# Autodesk Inventor assembly: gearLockAssembly
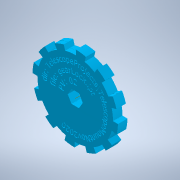
[picture p0: Inventor's stored thumbnail of the model, 180x180]
Saved by Autodesk Inventor 2021.2 (Build 252289000, 289)
## iProperties
Created: 2021-03-15
Part Number: gearLockAssembly
Document SubType Name: Assembly
Designer: robst
Author: robst
## Documents named in this file (4)
- C:\git\CAD-Development\robSteele\ShapeWays\TelescopeProjects\TelescopeMountNov2020\gearLockAssembly.iam
- C:\git\CAD-Development\robSteele\ShapeWays\TelescopeProjects\TelescopeMountNov2020\gearLockTopHalf.ipt
- C:\Users\robst\Documents\Inventor\Content Center Files\R2021\en-US\ANSI B18.3(03)\ANSI B18.3 - 10-32 UNF - UNF - 1(1).ipt
- C:\git\CAD-Development\robSteele\ShapeWays\TelescopeProjects\TelescopeMountNov2020\gearLockBottomHalf.ipt
## Components (3 placed, 3 different names)
1. gearLockTopHalf:1 — Flush:1, Tangent:1, Mate:1, Mate:2
2. Hexagon Socket Button Head Cap Screw - Inch No. 10-32 - 1:1 — Flush:1, Tangent:1
3. gearLockBottomHalf:1 — Mate:1, Mate:2
## Relationships (4: Mate 2, Flush 1, Tangent 1)
- Flush:1: gearLockTopHalf:1 ↔ Hexagon Socket Button Head Cap Screw - Inch No. 10-32 - 1:1
- Tangent:1 (0.508 mm): gearLockTopHalf:1 ↔ Hexagon Socket Button Head Cap Screw - Inch No. 10-32 - 1:1
- Mate:1: gearLockTopHalf:1 ↔ gearLockBottomHalf:1
- Mate:2: gearLockTopHalf:1 ↔ gearLockBottomHalf:1
